# Autodesk Inventor assembly: Ensamble eléctrico
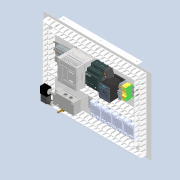
[picture p0: Inventor's stored thumbnail of the model, 180x180]
Saved by Autodesk Inventor 2021 (Build 250183000, 183)
## iProperties
Created: 2021-04-14
Part Number: Ensamble eléctrico
Document SubType Name: Assembly
Designer: Nelson
Mass: 3673.58 g
Surface Area: 11945 cm^2
Volume: 1889.25 cm^3
Density: 1.94447 g/cm^3
Author: Nelson
## Documents named in this file (20)
- E:\Documentos\Documentos\Michael_Rodriguez\Universidad_Nacional\Doceaba matricula\PAI\Proyecto PAI\Proyecto_PAI_2021\01 CAD\Ensamble eléctrico.iam
- E:\Documentos\Documentos\Michael_Rodriguez\Universidad_Nacional\Doceaba matricula\PAI\Proyecto PAI\Proyecto_PAI_2021\01 CAD\PLC-CP1E_N20DT1_D.iam
- E:\Documentos\Documentos\Michael_Rodriguez\Universidad_Nacional\Doceaba matricula\PAI\Proyecto PAI\Proyecto_PAI_2021\01 CAD\FuenteDC.iam
- E:\Documentos\Documentos\Michael_Rodriguez\Universidad_Nacional\Doceaba matricula\PAI\Proyecto PAI\Proyecto_PAI_2021\01 CAD\Rele de estado solido.ipt
- E:\Documentos\Documentos\Michael_Rodriguez\Universidad_Nacional\Doceaba matricula\PAI\Proyecto PAI\Proyecto_PAI_2021\01 CAD\Portafusible para fusible de 2A.ipt
- E:\Documentos\Documentos\Michael_Rodriguez\Universidad_Nacional\Doceaba matricula\PAI\Proyecto PAI\Proyecto_PAI_2021\01 CAD\Contactor.ipt
- E:\Documentos\Documentos\Michael_Rodriguez\Universidad_Nacional\Doceaba matricula\PAI\Proyecto PAI\Proyecto_PAI_2021\01 CAD\Riel 35x7.5 378mm.ipt
- E:\Documentos\Documentos\Michael_Rodriguez\Universidad_Nacional\Doceaba matricula\PAI\Proyecto PAI\Proyecto_PAI_2021\01 CAD\Bornera_AC.ipt
- E:\Documentos\Documentos\Michael_Rodriguez\Universidad_Nacional\Doceaba matricula\PAI\Proyecto PAI\Proyecto_PAI_2021\01 CAD\Bornera_DC.ipt
- E:\Documentos\Documentos\Michael_Rodriguez\Universidad_Nacional\Doceaba matricula\PAI\Proyecto PAI\Proyecto_PAI_2021\01 CAD\Bornera_Tierra.ipt
- E:\Documentos\Documentos\Michael_Rodriguez\Universidad_Nacional\Doceaba matricula\PAI\Proyecto PAI\Proyecto_PAI_2021\01 CAD\Canaleta 30x30 438mm.iam
- E:\Documentos\Documentos\Michael_Rodriguez\Universidad_Nacional\Doceaba matricula\PAI\Proyecto PAI\Proyecto_PAI_2021\01 CAD\Canaleta 30x30 378mm.iam
- E:\Documentos\Documentos\Michael_Rodriguez\Universidad_Nacional\Doceaba matricula\PAI\Proyecto PAI\Proyecto_PAI_2021\01 CAD\Canaleta 30x30 317mm.iam
- E:\Documentos\Documentos\Michael_Rodriguez\Universidad_Nacional\Doceaba matricula\PAI\Proyecto PAI\Proyecto_PAI_2021\01 CAD\Tapa_interior_1b.ipt
- E:\Documentos\Documentos\Michael_Rodriguez\Universidad_Nacional\Doceaba matricula\PAI\Proyecto PAI\Proyecto_PAI_2021\01 CAD\DIN EN ISO 7049 - ST4,8 x 13 - C - H.ipt
- E:\Documentos\Documentos\Michael_Rodriguez\Universidad_Nacional\Doceaba matricula\PAI\Proyecto PAI\Proyecto_PAI_2021\01 CAD\Ensamble electroválvula y bobina.iam
- E:\Documentos\Documentos\Michael_Rodriguez\Universidad_Nacional\Doceaba matricula\PAI\Proyecto PAI\Proyecto_PAI_2021\01 CAD\Fusible de 2A.ipt
- E:\Documentos\Documentos\Michael_Rodriguez\Universidad_Nacional\Doceaba matricula\PAI\Proyecto PAI\Proyecto_PAI_2021\01 CAD\Base Valvula.ipt
- E:\Documentos\Documentos\Michael_Rodriguez\Universidad_Nacional\Doceaba matricula\PAI\Proyecto PAI\Proyecto_PAI_2021\01 CAD\DIN EN ISO 7049 - ST4,8 x 38 - C - H.ipt
- C:\Users\Admin\Documents\Inventor\Content Center Files\R2021\es-ES\Parker Hose Barb 90deg Elbow to Male Pipe 129HB\Parker Hose Barb 90° Elbow to Male Pipe 129HB 129HB-4-4.ipt
## Components (65 placed, 19 different names)
1. PLC-CP1E_N20DT1_D:1 [sub-assembly] — Mate:13, Mate:14, Mate:147, Mate:148
2. FuenteDC:1 [sub-assembly] — Mate:15, Mate:16, Mate:148, Mate:149
3. Portafusible para fusible de 2A:1 — Mate:17, Mate:18, Mate:149, Mate:150, Mate:204, Mate:205
4. Contactor:1 — Mate:19, Mate:20, Mate:150, Mate:151
5. Riel 35x7.5 378mm:1 — Mate:13, Mate:14, Mate:15, Mate:16, Mate:17, Mate:18, Mate:19, Mate:20, Mate:21, Mate:22, Mate:23, Mate:24, Mate:26, Mate:27, Mate:28, Mate:29, Mate:31, Mate:32, Mate:34, Mate:35, Mate:37, Mate:38, Mate:39, Mate:40, Mate:42, Mate:43, Mate:45, Mate:46, Mate:48, Mate:49, Mate:51, Mate:52, Mate:53, Mate:54, Mate:56, Mate:57, Mate:87, Mate:96, Mate:97, Flush:45, Mate:141, Mate:143, Mate:145
6. Bornera_AC:1 — Mate:21, Mate:22, Mate:25, Mate:151
7. Bornera_AC:2 — Mate:23, Mate:24, Mate:25, Mate:65
8. Bornera_DC:1 — Mate:26, Mate:27, Mate:30, Mate:89
9. Bornera_DC:2 — Mate:28, Mate:29, Mate:30, Mate:33
10. Bornera_DC:3 — Mate:31, Mate:32, Mate:33, Mate:36
11. Bornera_DC:4 — Mate:34, Mate:35, Mate:36, Mate:146
12. Bornera_DC:5 — Mate:39, Mate:40, Mate:41, Mate:44
13. Bornera_DC:6 — Mate:42, Mate:43, Mate:44, Mate:47
14. Bornera_DC:7 — Mate:45, Mate:46, Mate:47, Mate:50
15. Bornera_DC:8 — Mate:48, Mate:49, Mate:50, Mate:89
16. Bornera_DC:9 — Mate:37, Mate:38, Mate:41, Mate:147
17. Bornera_Tierra:1 — Mate:51, Mate:52, Mate:55, Mate:65
18. Bornera_Tierra:2 — Mate:53, Mate:54, Mate:55, Mate:58
19. Bornera_Tierra:3 — Mate:56, Mate:57, Mate:58
20. Canaleta 30x30 438mm:1 [sub-assembly] — Mate:79, Mate:83, Mate:96, Flush:41, Mate:109, Flush:53, Mate:116, Mate:117, Mate:118, Mate:119, Mate:120, Mate:121
21. Canaleta 30x30 317mm:1 [sub-assembly] — Mate:79, Mate:81, Mate:87, Mate:94, Flush:41, Flush:42, Flush:54, Mate:110, Mate:111, Mate:112, Mate:113, Mate:114, Mate:115, Mate:146
22. Canaleta 30x30 438mm:2 [sub-assembly] — Mate:81, Mate:84, Flush:42, Flush:43, Mate:128, Mate:129, Mate:130, Mate:131, Mate:132, Mate:133
23. Canaleta 30x30 317mm:2 [sub-assembly] — Mate:83, Mate:84, Flush:43, Flush:44, Flush:45, Mate:122, Mate:123, Mate:124, Mate:125, Mate:126, Mate:127
24. Canaleta 30x30 378mm:1 [sub-assembly] — Mate:94, Mate:97, Flush:44, Mate:134, Mate:135, Mate:136, Mate:137, Mate:138, Mate:139
25. DIN EN ISO 7049 - C-H ST4,8 x 13 - C - H:1 — Mate:110, Mate:111
26. DIN EN ISO 7049 - C-H ST4,8 x 13 - C - H:2 — Mate:112, Mate:113
27. DIN EN ISO 7049 - C-H ST4,8 x 13 - C - H:3 — Mate:114, Mate:115
28. DIN EN ISO 7049 - C-H ST4,8 x 13 - C - H:4 — Mate:122, Mate:123
29. DIN EN ISO 7049 - C-H ST4,8 x 13 - C - H:5 — Mate:124, Mate:125
30. DIN EN ISO 7049 - C-H ST4,8 x 13 - C - H:6 — Mate:126, Mate:127
31. DIN EN ISO 7049 - C-H ST4,8 x 13 - C - H:7 — Mate:132, Mate:133
32. DIN EN ISO 7049 - C-H ST4,8 x 13 - C - H:8 — Mate:130, Mate:131
33. DIN EN ISO 7049 - C-H ST4,8 x 13 - C - H:9 — Mate:128, Mate:129
34. DIN EN ISO 7049 - C-H ST4,8 x 13 - C - H:10 — Mate:116, Mate:117
35. DIN EN ISO 7049 - C-H ST4,8 x 13 - C - H:11 — Mate:118, Mate:119
36. DIN EN ISO 7049 - C-H ST4,8 x 13 - C - H:12 — Mate:120, Mate:121
37. DIN EN ISO 7049 - C-H ST4,8 x 13 - C - H:13 — Mate:138, Mate:139
38. DIN EN ISO 7049 - C-H ST4,8 x 13 - C - H:14 — Mate:136, Mate:137
39. DIN EN ISO 7049 - C-H ST4,8 x 13 - C - H:15 — Mate:134, Mate:135
40. DIN EN ISO 7049 - C-H ST4,8 x 13 - C - H:16 — Mate:140, Mate:141
41. DIN EN ISO 7049 - C-H ST4,8 x 13 - C - H:17 — Mate:143
42. DIN EN ISO 7049 - C-H ST4,8 x 13 - C - H:18 — Mate:145
43. Rele de estado solido:1 — Mate:177, Mate:178, Mate:179, Mate:189, Mate:190, Mate:191, Mate:192, Nivelación:55
44. Rele de estado solido:2 — Mate:180, Mate:181, Mate:182, Mate:193, Mate:194, Mate:195
45. Rele de estado solido:3 — Mate:183, Mate:184, Mate:185, Mate:196, Mate:197, Mate:198, Mate:199
46. Rele de estado solido:4 — Mate:186, Mate:187, Mate:188, Mate:200, Mate:201, Mate:202, Mate:203
47. DIN EN ISO 7049 - C-H ST4,8 x 13 - C - H:19 — Mate:189, Mate:190
48. DIN EN ISO 7049 - C-H ST4,8 x 13 - C - H:20 — Mate:191, Mate:192
49. DIN EN ISO 7049 - C-H ST4,8 x 13 - C - H:21 — Mate:193, Mate:194
50. DIN EN ISO 7049 - C-H ST4,8 x 13 - C - H:22 — Mate:195
51. DIN EN ISO 7049 - C-H ST4,8 x 13 - C - H:23 — Mate:196, Mate:197
52. DIN EN ISO 7049 - C-H ST4,8 x 13 - C - H:24 — Mate:198, Mate:199
53. DIN EN ISO 7049 - C-H ST4,8 x 13 - C - H:25 — Mate:200, Mate:201
54. DIN EN ISO 7049 - C-H ST4,8 x 13 - C - H:26 — Mate:202, Mate:203
55. Fusible de 2A:1 — Mate:204, Mate:205
56. Ensamble electroválvula y bobina:2 [sub-assembly] — Coincidencia:207, Nivelación:56, Coincidencia:208, De rotación:5, De rotación:6, De rotación:7
57. Base Valvula:1 — Coincidencia:206, Nivelación:55, Coincidencia:207, Nivelación:56, Coincidencia:208, De rotación:1, De rotación:2, De rotación:3, De rotación:4
58. DIN EN ISO 7049 - C-H ST4,8 x 13 - C - H:27 — De rotación:1
59. DIN EN ISO 7049 - C-H ST4,8 x 13 - C - H:28 — De rotación:2
60. DIN EN ISO 7049 - C-H ST4,8 x 13 - C - H:29 — De rotación:4
61. DIN EN ISO 7049 - C-H ST4,8 x 13 - C - H:30 — De rotación:3
62. DIN EN ISO 7049 - C-H ST4,8 x 38 - C - H:1 — De rotación:6
63. DIN EN ISO 7049 - C-H ST4,8 x 38 - C - H:2 — De rotación:5
64. Terminación de manguera para tubería macho 129HB de Parker - Codo de 90° 129HB-4-4:1 — De rotación:7
65. Tapa_interior_1b:1 — Flush:51, Flush:52, Mate:109, Flush:53, Flush:54, Mate:140, Mate:177, Mate:178, Mate:179, Mate:180, Mate:181, Mate:182, Mate:183, Mate:184, Mate:185, Mate:186, Mate:187, Mate:188, Coincidencia:206
## Relationships (147: Mate 129, Flush 11, RevoluteJoint 7)
- Mate:13: PLC-CP1E_N20DT1_D:1 ↔ Riel 35x7.5 378mm:1
- Mate:14: PLC-CP1E_N20DT1_D:1 ↔ Riel 35x7.5 378mm:1
- Mate:15: FuenteDC:1 ↔ Riel 35x7.5 378mm:1
- Mate:16: FuenteDC:1 ↔ Riel 35x7.5 378mm:1
- Mate:17: Portafusible para fusible de 2A:1 ↔ Riel 35x7.5 378mm:1
- Mate:18: Portafusible para fusible de 2A:1 ↔ Riel 35x7.5 378mm:1
- Mate:19: Contactor:1 ↔ Riel 35x7.5 378mm:1
- Mate:20: Contactor:1 ↔ Riel 35x7.5 378mm:1
- Mate:21: Riel 35x7.5 378mm:1 ↔ Bornera_AC:1
- Mate:22: Riel 35x7.5 378mm:1 ↔ Bornera_AC:1
- Mate:23: Riel 35x7.5 378mm:1 ↔ Bornera_AC:2
- Mate:24: Riel 35x7.5 378mm:1 ↔ Bornera_AC:2
- Mate:25: Bornera_AC:1 ↔ Bornera_AC:2
- Mate:26: Riel 35x7.5 378mm:1 ↔ Bornera_DC:1
- Mate:27: Riel 35x7.5 378mm:1 ↔ Bornera_DC:1
- Mate:28: Riel 35x7.5 378mm:1 ↔ Bornera_DC:2
- Mate:29: Riel 35x7.5 378mm:1 ↔ Bornera_DC:2
- Mate:30: Bornera_DC:1 ↔ Bornera_DC:2
- Mate:31: Riel 35x7.5 378mm:1 ↔ Bornera_DC:3
- Mate:32: Riel 35x7.5 378mm:1 ↔ Bornera_DC:3
- Mate:33: Bornera_DC:2 ↔ Bornera_DC:3
- Mate:34: Riel 35x7.5 378mm:1 ↔ Bornera_DC:4
- Mate:35: Riel 35x7.5 378mm:1 ↔ Bornera_DC:4
- Mate:36: Bornera_DC:3 ↔ Bornera_DC:4
- Mate:37: Riel 35x7.5 378mm:1 ↔ Bornera_DC:9
- Mate:38: Riel 35x7.5 378mm:1 ↔ Bornera_DC:9
- Mate:39: Riel 35x7.5 378mm:1 ↔ Bornera_DC:5
- Mate:40: Riel 35x7.5 378mm:1 ↔ Bornera_DC:5
- Mate:41: Bornera_DC:5 ↔ Bornera_DC:9
- Mate:42: Riel 35x7.5 378mm:1 ↔ Bornera_DC:6
- Mate:43: Riel 35x7.5 378mm:1 ↔ Bornera_DC:6
- Mate:44: Bornera_DC:5 ↔ Bornera_DC:6
- Mate:45: Riel 35x7.5 378mm:1 ↔ Bornera_DC:7
- Mate:46: Riel 35x7.5 378mm:1 ↔ Bornera_DC:7
- Mate:47: Bornera_DC:6 ↔ Bornera_DC:7
- Mate:48: Riel 35x7.5 378mm:1 ↔ Bornera_DC:8
- Mate:49: Riel 35x7.5 378mm:1 ↔ Bornera_DC:8
- Mate:50: Bornera_DC:7 ↔ Bornera_DC:8
- Mate:51: Riel 35x7.5 378mm:1 ↔ Bornera_Tierra:1
- Mate:52: Riel 35x7.5 378mm:1 ↔ Bornera_Tierra:1
- Mate:53: Riel 35x7.5 378mm:1 ↔ Bornera_Tierra:2
- Mate:54: Riel 35x7.5 378mm:1 ↔ Bornera_Tierra:2
- Mate:55: Bornera_Tierra:1 ↔ Bornera_Tierra:2
- Mate:56: Riel 35x7.5 378mm:1 ↔ Bornera_Tierra:3
- Mate:57: Riel 35x7.5 378mm:1 ↔ Bornera_Tierra:3
- Mate:58: Bornera_Tierra:2 ↔ Bornera_Tierra:3
- Mate:65 (2 mm): Bornera_AC:2 ↔ Bornera_Tierra:1
- Mate:79: Canaleta 30x30 438mm:1 ↔ Canaleta 30x30 317mm:1
- Mate:81: Canaleta 30x30 317mm:1 ↔ Canaleta 30x30 438mm:2
- Mate:83: Canaleta 30x30 438mm:1 ↔ Canaleta 30x30 317mm:2
- Mate:84: Canaleta 30x30 438mm:2 ↔ Canaleta 30x30 317mm:2
- Mate:87: Riel 35x7.5 378mm:1 ↔ Canaleta 30x30 317mm:1
- Mate:89 (2 mm): Bornera_DC:1 ↔ Bornera_DC:8
- Mate:94: Canaleta 30x30 317mm:1 ↔ Canaleta 30x30 378mm:1
- Mate:96 (47 mm): Riel 35x7.5 378mm:1 ↔ Canaleta 30x30 438mm:1
- Mate:97 (48 mm): Riel 35x7.5 378mm:1 ↔ Canaleta 30x30 378mm:1
- Flush:41: Canaleta 30x30 438mm:1 ↔ Canaleta 30x30 317mm:1
- Flush:42: Canaleta 30x30 317mm:1 ↔ Canaleta 30x30 438mm:2
- Flush:43: Canaleta 30x30 438mm:2 ↔ Canaleta 30x30 317mm:2
- Flush:44: Canaleta 30x30 317mm:2 ↔ Canaleta 30x30 378mm:1
- Flush:45: Riel 35x7.5 378mm:1 ↔ Canaleta 30x30 317mm:2
- Flush:51: Tapa_interior_1b:1
- Flush:52: Tapa_interior_1b:1
- Mate:109: Canaleta 30x30 438mm:1 ↔ Tapa_interior_1b:1
- Flush:53 (10.29 mm): Canaleta 30x30 438mm:1 ↔ Tapa_interior_1b:1
- Flush:54 (21 mm): Canaleta 30x30 317mm:1 ↔ Tapa_interior_1b:1
- Mate:110: Canaleta 30x30 317mm:1 ↔ DIN EN ISO 7049 - C-H ST4,8 x 13 - C - H:1
- Mate:111: Canaleta 30x30 317mm:1 ↔ DIN EN ISO 7049 - C-H ST4,8 x 13 - C - H:1
- Mate:112: Canaleta 30x30 317mm:1 ↔ DIN EN ISO 7049 - C-H ST4,8 x 13 - C - H:2
- Mate:113: Canaleta 30x30 317mm:1 ↔ DIN EN ISO 7049 - C-H ST4,8 x 13 - C - H:2
- Mate:114: Canaleta 30x30 317mm:1 ↔ DIN EN ISO 7049 - C-H ST4,8 x 13 - C - H:3
- Mate:115: Canaleta 30x30 317mm:1 ↔ DIN EN ISO 7049 - C-H ST4,8 x 13 - C - H:3
- Mate:116: Canaleta 30x30 438mm:1 ↔ DIN EN ISO 7049 - C-H ST4,8 x 13 - C - H:10
- Mate:117: Canaleta 30x30 438mm:1 ↔ DIN EN ISO 7049 - C-H ST4,8 x 13 - C - H:10
- Mate:118: Canaleta 30x30 438mm:1 ↔ DIN EN ISO 7049 - C-H ST4,8 x 13 - C - H:11
- Mate:119: Canaleta 30x30 438mm:1 ↔ DIN EN ISO 7049 - C-H ST4,8 x 13 - C - H:11
- Mate:120: Canaleta 30x30 438mm:1 ↔ DIN EN ISO 7049 - C-H ST4,8 x 13 - C - H:12
- Mate:121: Canaleta 30x30 438mm:1 ↔ DIN EN ISO 7049 - C-H ST4,8 x 13 - C - H:12
- Mate:122: Canaleta 30x30 317mm:2 ↔ DIN EN ISO 7049 - C-H ST4,8 x 13 - C - H:4
- Mate:123: Canaleta 30x30 317mm:2 ↔ DIN EN ISO 7049 - C-H ST4,8 x 13 - C - H:4
- Mate:124: Canaleta 30x30 317mm:2 ↔ DIN EN ISO 7049 - C-H ST4,8 x 13 - C - H:5
- Mate:125: Canaleta 30x30 317mm:2 ↔ DIN EN ISO 7049 - C-H ST4,8 x 13 - C - H:5
- Mate:126: Canaleta 30x30 317mm:2 ↔ DIN EN ISO 7049 - C-H ST4,8 x 13 - C - H:6
- Mate:127: Canaleta 30x30 317mm:2 ↔ DIN EN ISO 7049 - C-H ST4,8 x 13 - C - H:6
- Mate:128: Canaleta 30x30 438mm:2 ↔ DIN EN ISO 7049 - C-H ST4,8 x 13 - C - H:9
- Mate:129: Canaleta 30x30 438mm:2 ↔ DIN EN ISO 7049 - C-H ST4,8 x 13 - C - H:9
- Mate:130: Canaleta 30x30 438mm:2 ↔ DIN EN ISO 7049 - C-H ST4,8 x 13 - C - H:8
- Mate:131: Canaleta 30x30 438mm:2 ↔ DIN EN ISO 7049 - C-H ST4,8 x 13 - C - H:8
- Mate:132: Canaleta 30x30 438mm:2 ↔ DIN EN ISO 7049 - C-H ST4,8 x 13 - C - H:7
- Mate:133: Canaleta 30x30 438mm:2 ↔ DIN EN ISO 7049 - C-H ST4,8 x 13 - C - H:7
- Mate:134: Canaleta 30x30 378mm:1 ↔ DIN EN ISO 7049 - C-H ST4,8 x 13 - C - H:15
- Mate:135: Canaleta 30x30 378mm:1 ↔ DIN EN ISO 7049 - C-H ST4,8 x 13 - C - H:15
- Mate:136: Canaleta 30x30 378mm:1 ↔ DIN EN ISO 7049 - C-H ST4,8 x 13 - C - H:14
- Mate:137: Canaleta 30x30 378mm:1 ↔ DIN EN ISO 7049 - C-H ST4,8 x 13 - C - H:14
- Mate:138: Canaleta 30x30 378mm:1 ↔ DIN EN ISO 7049 - C-H ST4,8 x 13 - C - H:13
- Mate:139: Canaleta 30x30 378mm:1 ↔ DIN EN ISO 7049 - C-H ST4,8 x 13 - C - H:13
- Mate:140: DIN EN ISO 7049 - C-H ST4,8 x 13 - C - H:16 ↔ Tapa_interior_1b:1
- Mate:141: Riel 35x7.5 378mm:1 ↔ DIN EN ISO 7049 - C-H ST4,8 x 13 - C - H:16
- Mate:143: Riel 35x7.5 378mm:1 ↔ DIN EN ISO 7049 - C-H ST4,8 x 13 - C - H:17
- Mate:145: Riel 35x7.5 378mm:1 ↔ DIN EN ISO 7049 - C-H ST4,8 x 13 - C - H:18
- Mate:146 (35 mm): Bornera_DC:4 ↔ Canaleta 30x30 317mm:1
- Mate:147 (5 mm): PLC-CP1E_N20DT1_D:1 ↔ Bornera_DC:9
- Mate:148 (11 mm): PLC-CP1E_N20DT1_D:1 ↔ FuenteDC:1
- Mate:149 (5 mm): FuenteDC:1 ↔ Portafusible para fusible de 2A:1
- Mate:150 (5 mm): Portafusible para fusible de 2A:1 ↔ Contactor:1
- Mate:151 (5 mm): Contactor:1 ↔ Bornera_AC:1
- Mate:177: Rele de estado solido:1 ↔ Tapa_interior_1b:1
- Mate:178: Rele de estado solido:1 ↔ Tapa_interior_1b:1
- Mate:179: Rele de estado solido:1 ↔ Tapa_interior_1b:1
- Mate:180: Rele de estado solido:2 ↔ Tapa_interior_1b:1
- Mate:181: Rele de estado solido:2 ↔ Tapa_interior_1b:1
- Mate:182: Rele de estado solido:2 ↔ Tapa_interior_1b:1
- Mate:183: Rele de estado solido:3 ↔ Tapa_interior_1b:1
- Mate:184: Rele de estado solido:3 ↔ Tapa_interior_1b:1
- Mate:185: Rele de estado solido:3 ↔ Tapa_interior_1b:1
- Mate:186: Rele de estado solido:4 ↔ Tapa_interior_1b:1
- Mate:187: Rele de estado solido:4 ↔ Tapa_interior_1b:1
- Mate:188: Rele de estado solido:4 ↔ Tapa_interior_1b:1
- Mate:189: Rele de estado solido:1 ↔ DIN EN ISO 7049 - C-H ST4,8 x 13 - C - H:19
- Mate:190: Rele de estado solido:1 ↔ DIN EN ISO 7049 - C-H ST4,8 x 13 - C - H:19
- Mate:191: Rele de estado solido:1 ↔ DIN EN ISO 7049 - C-H ST4,8 x 13 - C - H:20
- Mate:192: Rele de estado solido:1 ↔ DIN EN ISO 7049 - C-H ST4,8 x 13 - C - H:20
- Mate:193: Rele de estado solido:2 ↔ DIN EN ISO 7049 - C-H ST4,8 x 13 - C - H:21
- Mate:194: Rele de estado solido:2 ↔ DIN EN ISO 7049 - C-H ST4,8 x 13 - C - H:21
- Mate:195: Rele de estado solido:2 ↔ DIN EN ISO 7049 - C-H ST4,8 x 13 - C - H:22
- Mate:196: Rele de estado solido:3 ↔ DIN EN ISO 7049 - C-H ST4,8 x 13 - C - H:23
- Mate:197: Rele de estado solido:3 ↔ DIN EN ISO 7049 - C-H ST4,8 x 13 - C - H:23
- Mate:198: Rele de estado solido:3 ↔ DIN EN ISO 7049 - C-H ST4,8 x 13 - C - H:24
- Mate:199: Rele de estado solido:3 ↔ DIN EN ISO 7049 - C-H ST4,8 x 13 - C - H:24
- Mate:200: Rele de estado solido:4 ↔ DIN EN ISO 7049 - C-H ST4,8 x 13 - C - H:25
- Mate:201: Rele de estado solido:4 ↔ DIN EN ISO 7049 - C-H ST4,8 x 13 - C - H:25
- Mate:202: Rele de estado solido:4 ↔ DIN EN ISO 7049 - C-H ST4,8 x 13 - C - H:26
- Mate:203: Rele de estado solido:4 ↔ DIN EN ISO 7049 - C-H ST4,8 x 13 - C - H:26
- Mate:204: Portafusible para fusible de 2A:1 ↔ Fusible de 2A:1
- Mate:205: Portafusible para fusible de 2A:1 ↔ Fusible de 2A:1
- Coincidencia:206 [Mate]: Base Valvula:1 ↔ Tapa_interior_1b:1
- Nivelación:55 [Flush]: Rele de estado solido:1 ↔ Base Valvula:1
- Coincidencia:207 [Mate]: Ensamble electroválvula y bobina:2 ↔ Base Valvula:1
- Nivelación:56 [Flush]: Ensamble electroválvula y bobina:2 ↔ Base Valvula:1
- Coincidencia:208 [Mate]: Ensamble electroválvula y bobina:2 ↔ Base Valvula:1
- De rotación:1 [RevoluteJoint]: Base Valvula:1 ↔ DIN EN ISO 7049 - C-H ST4,8 x 13 - C - H:27
- De rotación:2 [RevoluteJoint]: Base Valvula:1 ↔ DIN EN ISO 7049 - C-H ST4,8 x 13 - C - H:28
- De rotación:3 [RevoluteJoint]: Base Valvula:1 ↔ DIN EN ISO 7049 - C-H ST4,8 x 13 - C - H:30
- De rotación:4 [RevoluteJoint]: Base Valvula:1 ↔ DIN EN ISO 7049 - C-H ST4,8 x 13 - C - H:29
- De rotación:5 [RevoluteJoint]: Ensamble electroválvula y bobina:2 ↔ DIN EN ISO 7049 - C-H ST4,8 x 38 - C - H:2
- De rotación:6 [RevoluteJoint]: Ensamble electroválvula y bobina:2 ↔ DIN EN ISO 7049 - C-H ST4,8 x 38 - C - H:1
- De rotación:7 [RevoluteJoint]: Ensamble electroválvula y bobina:2 ↔ Terminación de manguera para tubería macho 129HB de Parker - Codo de 90° 129HB-4-4:1
